# Autodesk Inventor assembly: PLANTER BOX
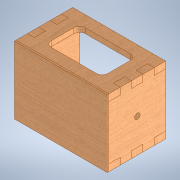
[picture p0: Inventor's stored thumbnail of the model, 180x180]
Saved by Autodesk Inventor 2021.2 (Build 252289000, 289)
## iProperties
Created: 2021-03-12
Part Number: PLANTER BOX
Document SubType Name: Assembly
Designer: 443201246
Author: 443201246
## Documents named in this file (5)
- C:\Users\443201246\Documents\8DT1\Planter Box\PLANTER BOX.iam
- C:\Users\443201246\Documents\8DT1\Planter Box\Parts\FRONT.ipt
- C:\Users\443201246\Documents\8DT1\Planter Box\Parts\SIDE.ipt
- C:\Users\443201246\Documents\8DT1\Planter Box\Parts\BACK.ipt
- C:\Users\443201246\Documents\8DT1\Planter Box\Parts\Base.ipt
## Components (5 placed, 2 different names)
1. FRONT:1 — Flush:1, Flush:2, Flush:3, Flush:4, Flush:5, Flush:6, Flush:11
2. FRONT:2 — Flush:1, Flush:2, Flush:3, Flush:7, Flush:8, Flush:9
3. FRONT:3 — Flush:4, Flush:5, Flush:6, Flush:10
4. FRONT:4 — Flush:7, Flush:8, Flush:9, Mate:1
5. Base:1 — Mate:1, Flush:10, Flush:11
## Relationships (12: Flush 11, Mate 1)
- Flush:1: FRONT:1 ↔ FRONT:2
- Flush:2: FRONT:1 ↔ FRONT:2
- Flush:3: FRONT:1 ↔ FRONT:2
- Flush:4: FRONT:1 ↔ FRONT:3
- Flush:5: FRONT:1 ↔ FRONT:3
- Flush:6: FRONT:1 ↔ FRONT:3
- Flush:7: FRONT:2 ↔ FRONT:4
- Flush:8: FRONT:2 ↔ FRONT:4
- Flush:9: FRONT:2 ↔ FRONT:4
- Mate:1: FRONT:4 ↔ Base:1
- Flush:10: FRONT:3 ↔ Base:1
- Flush:11: FRONT:1 ↔ Base:1
